# Autodesk Inventor assembly: 000 Ensamblaje 3d_LM-Welding_Tooling - BASIC
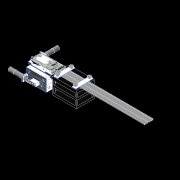
[picture p0: Inventor's stored thumbnail of the model, 180x180]
Saved by Autodesk Inventor 2018.3 (Build 223284000, 284)
## iProperties
Created: 2026-01-13
Part Number: 000 Ensamblaje 3d_LM-Welding_Tooling - BASIC
Document SubType Name: Assembly
Designer: aca6
Mass: 2650.67 g
Surface Area: 3394.3 cm^2
Volume: 1053.59 cm^3
Density: 2.51584 g/cm^3
Manufacturer-1: {"Name": "Embention Sistemas Inteligentes S.A.", "PartNumber": "3d_Welding_Tooling - BASIC", "Link": ""}
Manufacturer-2: {"Name": "", "PartNumber": "", "Link": ""}
Manufacturer-3: {"Name": "", "PartNumber": "", "Link": ""}
Manufacturer-4: {"Name": "", "PartNumber": "", "Link": ""}
Manufacturer-5: {"Name": "", "PartNumber": "", "Link": ""}
Provider-1: {"Name": "", "PartNumber": "", "Link": ""}
Provider-2: {"Name": "", "PartNumber": "", "Link": ""}
Provider-3: {"Name": "", "PartNumber": "", "Link": ""}
Provider-4: {"Name": "", "PartNumber": "", "Link": ""}
Provider-5: {"Name": "", "PartNumber": "", "Link": ""}
Author: aca6
## Documents named in this file (12)
- C:\Users\aca6\git\LM\items\3d_LM\items\LM-Welding_Tooling\3d_LM-Welding_Tooling\variants\BASIC\000 Ensamblaje 3d_LM-Welding_Tooling - BASIC.iam
- C:\Users\aca6\git\LM\items\3d_LM\items\LM-Welding_Tooling\3d_LM-Welding_Tooling\3d\3d_LM-Welding_Tooling - Welding Placement.ipt
- C:\Users\aca6\git\LM\items\3d_LM\items\LM-Welding_Tooling\3d_LM-Welding_Tooling\3d\3d_LM-Welding_Tooling - Wire.ipt
- C:\Users\aca6\git\LM\items\3d_LM\items\LM-Welding_Tooling\3d_LM-Welding_Tooling\3d\3d_LM-Welding_Tooling - Bot Wire.ipt
- C:\Users\aca6\git\LM\items\3d_LM\items\LM-Welding_Tooling\3d_LM-Welding_Tooling\3d\3d_LM-Welding_Tooling -  4x14 Guide Pin.ipt
- C:\Users\aca6\git\LM\items\3d_LM\items\LM-Welding_Tooling\3d_LM-Welding_Tooling\3d\3d_LM-Welding_Tooling -  Tab.ipt
- C:\Users\aca6\git\LM\items\_accesories\Tornilleria\Insertos\3d_Genéricos\3d\Inserto roscado M4x5.6x7.95.ipt
- C:\Users\aca6\git\LM\items\3d_LM\items\LM-Welding_Tooling\3d_LM-Welding_Tooling\3d\Knurled Screw_ Stainless Steel DIN 464-M4-10-A4.ipt
- C:\Users\aca6\git\LM\items\3d_LM\variants\BASIC\dummy\3d_LM - BASIC - welding tooling_dummy.ipt
- C:\Users\aca6\git\LM\items\3d_LM\3d\3d_LM - Bottom Wire - Phantom.ipt
- C:\Users\aca6\git\LM\items\3d_LM\3d\3d_LM - Top Wire - Phantom.ipt
- C:\Users\aca6\git\LM\items\3d_LM\items\LM-Welding_Tooling\3d_LM-Welding_Tooling\3d\3d_LM-Welding_Tooling - Lathe carriage.iam
## Components (19 placed, 11 different names)
1. 3d_LM-Welding_Tooling - Welding Placement:1 — Mate:126, Mate:127, Mate:128, Mate:129, Mate:130, Mate:131, Mate:136, Mate:137, Mate:204, Mate:205, Mate:206, Mate:207, Mate:208, Flush:141, Flush:142, Flush:143
2. 3d_LM-Welding_Tooling -  4x14 Guide Pin:1 — Mate:128, Mate:129
3. 3d_LM-Welding_Tooling -  4x14 Guide Pin:2 — Mate:126, Mate:127
4. 3d_LM-Welding_Tooling -  Tab:1 — Mate:130, Mate:131, Mate:217, Mate:223
5. 3d_LM-Welding_Tooling -  Tab:2 — Mate:136, Mate:137, Mate:219, Mate:221
6. Inserto roscado M4x5.6x7.95:1 — Mate:204, Mate:205, Mate:216
7. Inserto roscado M4x5.6x7.95:2 — Mate:207, Flush:143, Mate:218
8. Inserto roscado M4x5.6x7.95:3 — Mate:208, Flush:142, Mate:220
9. Inserto roscado M4x5.6x7.95:4 — Mate:206, Flush:141, Mate:222
10. Knurled Screw_ Stainless Steel DIN 464-M4-10-A4:1 — Mate:216, Mate:217
11. Knurled Screw_ Stainless Steel DIN 464-M4-10-A4:2 — Mate:222, Mate:223
12. Knurled Screw_ Stainless Steel DIN 464-M4-10-A4:3 — Mate:220, Mate:221
13. Knurled Screw_ Stainless Steel DIN 464-M4-10-A4:4 — Mate:218, Mate:219
14. 3d_LM - Top Wire - Phantom:1 — Mate:244, Mate:245, Mate:246, Mate:250, Mate:251, Mate:252
15. 3d_LM - Bottom Wire - Phantom:1 — Mate:241, Mate:242, Mate:243, Mate:247, Mate:248, Mate:249
16. 3d_LM - BASIC - welding tooling_dummy:1 — Mate:247, Mate:248, Mate:249, Mate:250, Mate:251, Mate:252, Mate:253, Mate:254, Mate:255
17. 3d_Welding_Tooling - Lathe carriage:1 [sub-assembly] — Mate:253, Mate:254, Mate:255
18. 3d_LM-Welding_Tooling - Wire:1 — Mate:244, Mate:245, Mate:246
19. 3d_LM-Welding_Tooling - Bot Wire:1 — Mate:241, Mate:242, Mate:243
## Relationships (39: Mate 36, Flush 3)
- Mate:126: 3d_LM-Welding_Tooling - Welding Placement:1 ↔ 3d_LM-Welding_Tooling -  4x14 Guide Pin:2
- Mate:127: 3d_LM-Welding_Tooling - Welding Placement:1 ↔ 3d_LM-Welding_Tooling -  4x14 Guide Pin:2
- Mate:128: 3d_LM-Welding_Tooling - Welding Placement:1 ↔ 3d_LM-Welding_Tooling -  4x14 Guide Pin:1
- Mate:129: 3d_LM-Welding_Tooling - Welding Placement:1 ↔ 3d_LM-Welding_Tooling -  4x14 Guide Pin:1
- Mate:130 (2.5 mm): 3d_LM-Welding_Tooling - Welding Placement:1 ↔ 3d_LM-Welding_Tooling -  Tab:1
- Mate:131: 3d_LM-Welding_Tooling - Welding Placement:1 ↔ 3d_LM-Welding_Tooling -  Tab:1
- Mate:136: 3d_LM-Welding_Tooling - Welding Placement:1 ↔ 3d_LM-Welding_Tooling -  Tab:2
- Mate:137 (2.5 mm): 3d_LM-Welding_Tooling - Welding Placement:1 ↔ 3d_LM-Welding_Tooling -  Tab:2
- Mate:204: 3d_LM-Welding_Tooling - Welding Placement:1 ↔ Inserto roscado M4x5.6x7.95:1
- Mate:205: 3d_LM-Welding_Tooling - Welding Placement:1 ↔ Inserto roscado M4x5.6x7.95:1
- Mate:206: 3d_LM-Welding_Tooling - Welding Placement:1 ↔ Inserto roscado M4x5.6x7.95:4
- Mate:207: 3d_LM-Welding_Tooling - Welding Placement:1 ↔ Inserto roscado M4x5.6x7.95:2
- Mate:208: 3d_LM-Welding_Tooling - Welding Placement:1 ↔ Inserto roscado M4x5.6x7.95:3
- Flush:141: 3d_LM-Welding_Tooling - Welding Placement:1 ↔ Inserto roscado M4x5.6x7.95:4
- Flush:142: 3d_LM-Welding_Tooling - Welding Placement:1 ↔ Inserto roscado M4x5.6x7.95:3
- Flush:143: 3d_LM-Welding_Tooling - Welding Placement:1 ↔ Inserto roscado M4x5.6x7.95:2
- Mate:216: Inserto roscado M4x5.6x7.95:1 ↔ Knurled Screw_ Stainless Steel DIN 464-M4-10-A4:1
- Mate:217: 3d_LM-Welding_Tooling -  Tab:1 ↔ Knurled Screw_ Stainless Steel DIN 464-M4-10-A4:1
- Mate:218: Inserto roscado M4x5.6x7.95:2 ↔ Knurled Screw_ Stainless Steel DIN 464-M4-10-A4:4
- Mate:219: 3d_LM-Welding_Tooling -  Tab:2 ↔ Knurled Screw_ Stainless Steel DIN 464-M4-10-A4:4
- Mate:220: Inserto roscado M4x5.6x7.95:3 ↔ Knurled Screw_ Stainless Steel DIN 464-M4-10-A4:3
- Mate:221: 3d_LM-Welding_Tooling -  Tab:2 ↔ Knurled Screw_ Stainless Steel DIN 464-M4-10-A4:3
- Mate:222: Inserto roscado M4x5.6x7.95:4 ↔ Knurled Screw_ Stainless Steel DIN 464-M4-10-A4:2
- Mate:223: 3d_LM-Welding_Tooling -  Tab:1 ↔ Knurled Screw_ Stainless Steel DIN 464-M4-10-A4:2
- Mate:241: 3d_LM - Bottom Wire - Phantom:1 ↔ 3d_LM-Welding_Tooling - Bot Wire:1
- Mate:242: 3d_LM - Bottom Wire - Phantom:1 ↔ 3d_LM-Welding_Tooling - Bot Wire:1
- Mate:243: 3d_LM - Bottom Wire - Phantom:1 ↔ 3d_LM-Welding_Tooling - Bot Wire:1
- Mate:244: 3d_LM - Top Wire - Phantom:1 ↔ 3d_LM-Welding_Tooling - Wire:1
- Mate:245: 3d_LM - Top Wire - Phantom:1 ↔ 3d_LM-Welding_Tooling - Wire:1
- Mate:246: 3d_LM - Top Wire - Phantom:1 ↔ 3d_LM-Welding_Tooling - Wire:1
- Mate:247: 3d_LM - Bottom Wire - Phantom:1 ↔ 3d_LM - BASIC - welding tooling_dummy:1
- Mate:248: 3d_LM - Bottom Wire - Phantom:1 ↔ 3d_LM - BASIC - welding tooling_dummy:1
- Mate:249 (-7 mm): 3d_LM - Bottom Wire - Phantom:1 ↔ 3d_LM - BASIC - welding tooling_dummy:1
- Mate:250: 3d_LM - Top Wire - Phantom:1 ↔ 3d_LM - BASIC - welding tooling_dummy:1
- Mate:251: 3d_LM - Top Wire - Phantom:1 ↔ 3d_LM - BASIC - welding tooling_dummy:1
- Mate:252 (-7 mm): 3d_LM - Top Wire - Phantom:1 ↔ 3d_LM - BASIC - welding tooling_dummy:1
- Mate:253: 3d_LM - BASIC - welding tooling_dummy:1 ↔ 3d_Welding_Tooling - Lathe carriage:1
- Mate:254: 3d_LM - BASIC - welding tooling_dummy:1 ↔ 3d_Welding_Tooling - Lathe carriage:1
- Mate:255: 3d_LM - BASIC - welding tooling_dummy:1 ↔ 3d_Welding_Tooling - Lathe carriage:1
